# Autodesk Inventor assembly: VersaPlanetary_v2_2 Stage_10_1_with_NEO 550
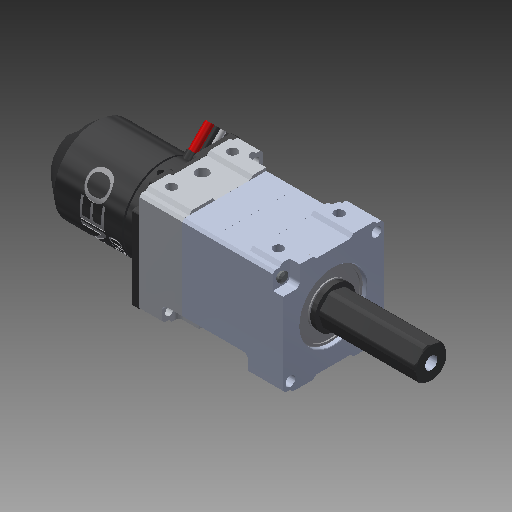
[picture p0: Inventor's stored thumbnail of the model, 512x512]
Saved by Autodesk Inventor 2018.3 (Build 223284000, 284)
## iProperties
Created: 2016-10-31
Part Number: VersaPlanetary_v2_2 Stage_10_1_with_NEO 550
Description: STEP AP214
Document SubType Name: Assembly
Designer: carls
Sending System: SolidWorks 2016
Preprocessor: SwSTEP 2.0
Title: 217-4973_1stage_550.STEP
Revision Number: ANY
## Documents named in this file (16)
- C:\Users\myerpaul\Documents\GrabCAD\Infinite Recharge 2020\Build season\VersaPlanetary_v2_2 Stage_10_1_with_NEO 550.iam
- C:\Users\myerpaul\Documents\GrabCAD\Infinite Recharge 2020\Build season\217-2625-026 Rev1.ipt
- C:\Users\myerpaul\Documents\GrabCAD\Infinite Recharge 2020\Build season\217-2742-001 Rev4.ipt
- C:\Users\myerpaul\Documents\GrabCAD\Infinite Recharge 2020\Build season\217-2625-017 Rev1_9714K61.ipt
- C:\Users\myerpaul\Documents\GrabCAD\Infinite Recharge 2020\Build season\217-2625-018 Rev1_98541A410.ipt
- C:\Users\myerpaul\Documents\GrabCAD\Infinite Recharge 2020\Build season\832-1750-Ring-Gear-Screw_SSA0832-0500ZC.ipt
- C:\Users\myerpaul\Documents\GrabCAD\Infinite Recharge 2020\Build season\217-2625-025 Rev1.ipt
- C:\Users\myerpaul\Documents\GrabCAD\Infinite Recharge 2020\Build season\217-4649-005 Rev1_SSA0003-008BA.ipt
- C:\Users\myerpaul\Documents\GrabCAD\Infinite Recharge 2020\Build season\217-2822-001 Rev4.ipt
- C:\Users\myerpaul\Documents\GrabCAD\Infinite Recharge 2020\Build season\217-2820 Rev1_Public.iam
- C:\Users\myerpaul\Documents\GrabCAD\Infinite Recharge 2020\Build season\217-2816-001 Rev1.ipt
- C:\Users\myerpaul\Documents\GrabCAD\Infinite Recharge 2020\Build season\217-4649-001 Rev1.ipt
- C:\Users\myerpaul\Documents\GrabCAD\Infinite Recharge 2020\Build season\217-4649-007 Rev1_94105A824.ipt
- C:\Users\myerpaul\Documents\GrabCAD\Infinite Recharge 2020\Build season\217-2625-012 Rev1.ipt
- C:\Users\myerpaul\Documents\GrabCAD\Infinite Recharge 2020\Build season\REV Neo 550.ipt
- C:\Users\myerpaul\Documents\GrabCAD\Infinite Recharge 2020\Build season\VersaPlanetary Output Shafts_0.500_ Hex (217-2615-003).iam
## Components (19 placed, 19 different names)
1. 217-2625-026 Rev1_1 — Insert:1, Flush:1
2. 217-2742-001 Rev4_2
3. 217-2742-001 Rev4_3 — Insert:7
4. 217-2625-017 Rev1_9714K61_4
5. 217-2625-018 Rev1_98541A410_6
6. 832-1750-Ring-Gear-Screw_SSA0832-0500ZC_7
7. 832-1750-Ring-Gear-Screw_SSA0832-0500ZC_8
8. 217-2625-025 Rev1_9 — Insert:3, Flush:3, Insert:4
9. 217-4649-005 Rev1_SSA0003-008BA_12
10. 217-4649-005 Rev1_SSA0003-008BA_13
11. 217-2822-001 Rev4_14 — Insert:4, Insert:6
12. 217-2820 Rev1_Public_16 [sub-assembly]
13. 217-2816-001 Rev1_17 — Insert:1, Flush:1, Insert:2, Flush:2
14. 217-4649-001 Rev1_18
15. 217-4649-007 Rev1_94105A824_19
16. 217-2625-012 Rev1_20
17. 217-2816-001 Rev1:2 — Insert:2, Flush:2, Insert:3, Flush:3
18. REV Neo 550:1 — Insert:6
19. VersaPlanetary Output Shafts_0.500_ Hex (217-2615-003):1 [sub-assembly] — Insert:7
## Relationships (9: Insert 6, Flush 3)
- Insert:1: 217-2625-026 Rev1_1 ↔ 217-2816-001 Rev1_17
- Flush:1: 217-2625-026 Rev1_1 ↔ 217-2816-001 Rev1_17
- Insert:2: 217-2816-001 Rev1_17 ↔ 217-2816-001 Rev1:2
- Flush:2: 217-2816-001 Rev1_17 ↔ 217-2816-001 Rev1:2
- Insert:3: 217-2625-025 Rev1_9 ↔ 217-2816-001 Rev1:2
- Flush:3: 217-2625-025 Rev1_9 ↔ 217-2816-001 Rev1:2
- Insert:4 (-1.778 mm): 217-2625-025 Rev1_9 ↔ 217-2822-001 Rev4_14
- Insert:6: 217-2822-001 Rev4_14 ↔ REV Neo 550:1
- Insert:7: 217-2742-001 Rev4_3 ↔ VersaPlanetary Output Shafts_0.500_ Hex (217-2615-003):1
